# Autodesk Inventor assembly: писюны_MIR2_MIR
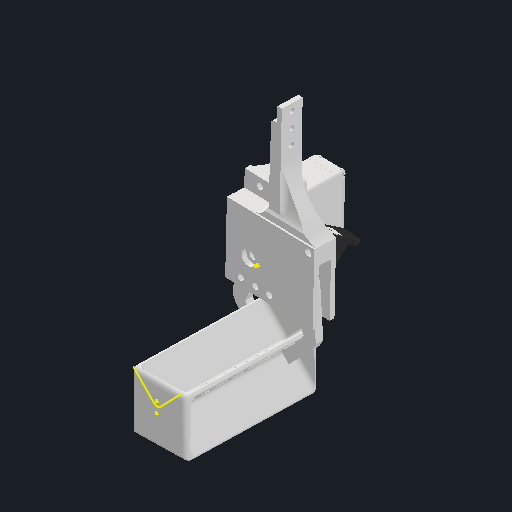
[picture p0: Inventor's stored thumbnail of the model, 512x512]
Saved by Autodesk Inventor 2025 (Build 290162000, 162)
## iProperties
Created: 2024-12-28
Part Number: писюны_MIR2_MIR
Document SubType Name: Assembly
Designer: GameHD
Author: Phantom
## Documents named in this file (9)
- C:\Users\Phantom\Desktop\Phantom16950\писюны_MIR2_MIR.iam
- C:\Users\Phantom\Desktop\Phantom16950\2000-0025-0002\2000-0025-0002_MIR4_MIR1_MIR.ipt
- C:\Users\GameHD\Downloads\Telegram Desktop\tetrix_metal_servo_horn\tetrix_metal_servo_horn_MIR1_MIR.ipt
- C:\Users\Phantom\Desktop\Phantom16950\держать писюны_MIR2_MIR.ipt
- C:\Users\Phantom\Desktop\Phantom16950\писюн 2_MIR4_MIR.ipt
- C:\Users\Phantom\Desktop\Phantom16950\писюн_MIR2_MIR.ipt
- C:\Users\Phantom\Desktop\Phantom16950\держать писюны 2ч_MIR1_MIR.ipt
- C:\Users\Phantom\Desktop\Phantom16950\am-5401 Sample.ipt
- C:\Users\Phantom\Downloads\Telegram Desktop\REV-31-1557\REV-31-1557.ipt
## Components (8 placed, 8 different names)
1. tetrix_metal_servo_horn_MIR1_MIR:1 — Совмещение:16, Совмещение:18, Совмещение:15, Совмещение:19
2. держать писюны_MIR2_MIR:1 — Совмещение:16, Заподлицо:1, Совмещение:14, Совмещение:18
3. писюн 2_MIR4_MIR:1 — Совмещение:18, Совмещение:12
4. писюн_MIR2_MIR:1 — Совмещение:15, Совмещение:19, Совмещение:21
5. держать писюны 2ч_MIR1_MIR:1 — Совмещение:21, Заподлицо:1, Совмещение:14
6. am-5401 Sample:1 — Совмещение:12
7. REV-31-1557:1
8. 2000-0025-0002_MIR4_MIR1_MIR:3 — Совмещение:18
## Relationships (9: Mate 8, Flush 1)
- Совмещение:16 [Mate]: tetrix_metal_servo_horn_MIR1_MIR:1 ↔ держать писюны_MIR2_MIR:1
- Совмещение:18 [Mate]: tetrix_metal_servo_horn_MIR1_MIR:1 ↔ писюн 2_MIR4_MIR:1
- Совмещение:15 [Mate]: tetrix_metal_servo_horn_MIR1_MIR:1 ↔ писюн_MIR2_MIR:1
- Совмещение:19 [Mate]: tetrix_metal_servo_horn_MIR1_MIR:1 ↔ писюн_MIR2_MIR:1
- Совмещение:21 [Mate]: писюн_MIR2_MIR:1 ↔ держать писюны 2ч_MIR1_MIR:1
- Заподлицо:1 [Flush]: держать писюны_MIR2_MIR:1 ↔ держать писюны 2ч_MIR1_MIR:1
- Совмещение:12 [Mate]: писюн 2_MIR4_MIR:1 ↔ am-5401 Sample:1
- Совмещение:14 [Mate]: держать писюны_MIR2_MIR:1 ↔ держать писюны 2ч_MIR1_MIR:1
- Совмещение:18 [Mate]: держать писюны_MIR2_MIR:1 ↔ 2000-0025-0002_MIR4_MIR1_MIR:3
